# Autodesk Inventor assembly: 42146-12
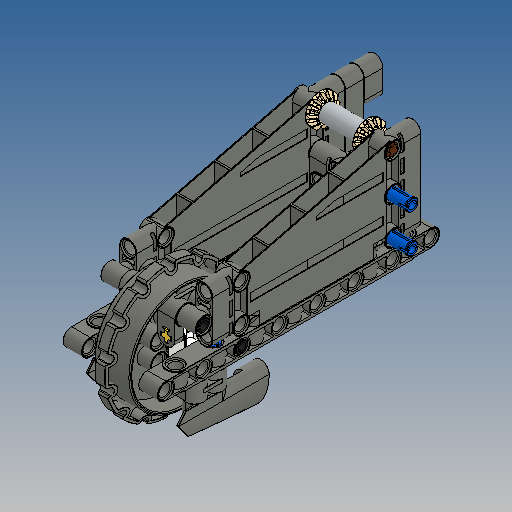
[picture p0: Inventor's stored thumbnail of the model, 512x512]
Saved by Autodesk Inventor 2025 (Build 290162010, 162A)
## iProperties
Created: 2024-11-18
Part Number: 42146-12
Material: Generisch
Document SubType Name: Assembly
Designer: hp.muther
Author: hp.muther
## Documents named in this file (20)
- D:\Inventor\Projekte\Muther\LEGO Technic\LEGO Technik - Raupenkran LR 13000 (42146)\42146-01-12.iam
- D:\Inventor\Projekte\Muther\LEGO Technic\LEGO Pieces\Paneelen\18945-DkBluishGray.ipt
- D:\Inventor\Projekte\Muther\LEGO Technic\LEGO Pieces\Pin's\2780-Black.ipt
- D:\Inventor\Projekte\Muther\LEGO Technic\LEGO Pieces\Pin's\11214-Red.ipt
- D:\Inventor\Projekte\Muther\LEGO Technic\LEGO Pieces\Pin's\6558-Blue.ipt
- D:\Inventor\Projekte\Muther\LEGO Technic\LEGO Pieces\Lochbalken\60483-DkBluishGray.ipt
- D:\Inventor\Projekte\Muther\LEGO Technic\LEGO Pieces\Lochbalken\32316-DkBluishGray.ipt
- D:\Inventor\Projekte\Muther\LEGO Technic\LEGO Pieces\Verbindungselemente\15100-DkBluishGray.ipt
- D:\Inventor\Projekte\Muther\LEGO Technic\LEGO Pieces\Achsen\4519-Yellow.ipt
- D:\Inventor\Projekte\Muther\LEGO Technic\LEGO Pieces\Verbindungselemente\41678-DkBluishGray.ipt
- D:\Inventor\Projekte\Muther\LEGO Technic\LEGO Pieces\Verbindungselemente\32184-White.ipt
- D:\Inventor\Projekte\Muther\LEGO Technic\LEGO Pieces\Achsen\24316-ReddishBrown.ipt
- D:\Inventor\Projekte\Muther\LEGO Technic\LEGO Pieces\Paneelen\11946-DkBluishGray.ipt
- D:\Inventor\Projekte\Muther\LEGO Technic\LEGO Pieces\Verbindungselemente\39793-DkBluishGray.ipt
- D:\Inventor\Projekte\Muther\LEGO Technic\LEGO Pieces\Achsen\15462-ReddishBrown.ipt
- D:\Inventor\Projekte\Muther\LEGO Technic\LEGO Pieces\Zahnrad\6589-Tan.ipt
- D:\Inventor\Projekte\Muther\LEGO Technic\LEGO Pieces\Rund\62462-LtBluishGray.ipt
- D:\Inventor\Projekte\Muther\LEGO Technic\LEGO Pieces\Lochbalken\771710-DkBluishGray.ipt
- D:\Inventor\Projekte\Muther\LEGO Technic\LEGO Pieces\Paneelen\11947-DkBluishGray.ipt
- D:\Inventor\Projekte\Muther\LEGO Technic\LEGO Pieces\Räder, Raupe\45229-DkBluishGray.ipt
## Components (48 placed, 19 different names)
1. 18945-DkBluishGray:1 — Einfügen:9, Passend:2, Einfügen:10, Einfügen:11, Einfügen:12, Einfügen:13, Winkel:1, Einfügen:29, Passend:8, Einfügen:31
2. 2780-Black:1 — Einfügen:6
3. 2780-Black:2 — Einfügen:8, Passend:2
4. 2780-Black:3 — Einfügen:11, Passend:3
5. 11214-Red:1 — Einfügen:5, Passend:1
6. 2780-Black:4 — Einfügen:12
7. 2780-Black:5 — Einfügen:14, Passend:14
8. 2780-Black:6 — Einfügen:22, Passend:7
9. 6558-Blue:1 — Einfügen:21
10. 6558-Blue:2 — Einfügen:26
11. 6558-Blue:3 — Einfügen:27
12. 6558-Blue:4 — Einfügen:28, Passend:8
13. 6558-Blue:5 — Einfügen:25, Passend:16
14. 2780-Black:7 — Einfügen:35
15. 2780-Black:8 — Einfügen:36, Passend:9
16. 2780-Black:9 — Einfügen:39, Passend:13
17. 2780-Black:10 — Einfügen:38
18. 2780-Black:11 — Einfügen:45, Passend:15
19. 6558-Blue:6 — Einfügen:44
20. 60483-DkBluishGray:1 — Einfügen:5, Einfügen:6, Einfügen:7
21. 32316-DkBluishGray:1 — Einfügen:7, Passend:1, Einfügen:8, Einfügen:9
22. 15100-DkBluishGray:1 — Einfügen:10, Einfügen:15, Winkel:1
23. 771710-DkBluishGray:1 — Einfügen:13, Passend:3, Einfügen:14, Einfügen:23
24. 2780-Black:12 — Einfügen:15
25. 4519-Yellow:1 — Einfügen:1, Passend:4, Passend:6
26. 41678-DkBluishGray:1 — Einfügen:1, Einfügen:16
27. 32184-White:1 — Einfügen:16, Passend:4, Passend:5, Einfügen:17, Einfügen:19, Passend:19
28. 4519-Yellow:2 — Passend:5
29. 41678-DkBluishGray:2 — Einfügen:17, Einfügen:18, Einfügen:23, Einfügen:24, Passend:7
30. 32184-White:2 — Einfügen:18, Passend:6, Passend:14
31. 24316-ReddishBrown:1 — Einfügen:19, Passend:17, Passend:18
32. 11946-DkBluishGray:1 — Einfügen:21, Einfügen:22, Einfügen:24
33. 39793-DkBluishGray:1 — Einfügen:25, Einfügen:26, Einfügen:27, Einfügen:28, Einfügen:29, Einfügen:47
34. 15462-ReddishBrown:1 — Einfügen:30, Einfügen:31
35. 6589-Tan:1 — Einfügen:30, Einfügen:32
36. 6589-Tan:2 — Einfügen:33
37. 62462-LtBluishGray:1 — Einfügen:32, Einfügen:33
38. 18945-DkBluishGray:2 — Einfügen:34, Winkel:2, Einfügen:35, Einfügen:36, Einfügen:37, Einfügen:47, Passend:16
39. 15100-DkBluishGray:2 — Einfügen:34, Winkel:2, Einfügen:38
40. 771710-DkBluishGray:2 — Einfügen:37, Passend:9, Einfügen:39, Einfügen:43, Pos. Zahnrad
41. 4519-Yellow:3 — Passend:10, Passend:12
42. 41678-DkBluishGray:3 — Einfügen:40
43. 4519-Yellow:4 — Passend:11
44. 41678-DkBluishGray:4 — Einfügen:41, Einfügen:42, Einfügen:43, Einfügen:46, Passend:15
45. 32184-White:4 — Einfügen:42, Passend:12, Passend:13
46. 32184-White:5 — Passend:10, Einfügen:40, Passend:11, Einfügen:41
47. 11947-DkBluishGray:1 — Einfügen:44, Einfügen:45, Einfügen:46
48. 45229-DkBluishGray:1 — Passend:17, Passend:18, Passend:19, Pos. Zahnrad
## Relationships (68: Insert 46, Mate 20, Angle 2)
- Pos. Zahnrad [Mate] (12.659 mm): 771710-DkBluishGray:2 ↔ 45229-DkBluishGray:1
- Einfügen:1 [Insert]: 4519-Yellow:1 ↔ 41678-DkBluishGray:1
- [Insert]: 4519-Yellow:2 ↔ 41678-DkBluishGray:2
- [Insert]: 4519-Yellow:3 ↔ 41678-DkBluishGray:3
- [Insert]: 4519-Yellow:4 ↔ 41678-DkBluishGray:4
- Einfügen:5 [Insert]: 11214-Red:1 ↔ 60483-DkBluishGray:1
- Einfügen:6 [Insert]: 2780-Black:1 ↔ 60483-DkBluishGray:1
- Einfügen:7 [Insert]: 60483-DkBluishGray:1 ↔ 32316-DkBluishGray:1
- Passend:1 [Mate]: 11214-Red:1 ↔ 32316-DkBluishGray:1
- Einfügen:8 [Insert]: 2780-Black:2 ↔ 32316-DkBluishGray:1
- Einfügen:9 [Insert]: 18945-DkBluishGray:1 ↔ 32316-DkBluishGray:1
- Passend:2 [Mate]: 18945-DkBluishGray:1 ↔ 2780-Black:2
- Einfügen:10 [Insert]: 18945-DkBluishGray:1 ↔ 15100-DkBluishGray:1
- Einfügen:11 [Insert]: 18945-DkBluishGray:1 ↔ 2780-Black:3
- Einfügen:12 [Insert]: 18945-DkBluishGray:1 ↔ 2780-Black:4
- Einfügen:13 [Insert]: 18945-DkBluishGray:1 ↔ 771710-DkBluishGray:1
- Passend:3 [Mate]: 2780-Black:3 ↔ 771710-DkBluishGray:1
- Einfügen:14 [Insert]: 2780-Black:5 ↔ 771710-DkBluishGray:1
- Einfügen:15 [Insert]: 15100-DkBluishGray:1 ↔ 2780-Black:12
- Einfügen:16 [Insert]: 41678-DkBluishGray:1 ↔ 32184-White:1
- Passend:4 [Mate]: 4519-Yellow:1 ↔ 32184-White:1
- Passend:5 [Mate]: 32184-White:1 ↔ 4519-Yellow:2
- Einfügen:17 [Insert]: 32184-White:1 ↔ 41678-DkBluishGray:2
- Einfügen:18 [Insert]: 41678-DkBluishGray:2 ↔ 32184-White:2
- Passend:6 [Mate]: 4519-Yellow:1 ↔ 32184-White:2
- Einfügen:19 [Insert]: 32184-White:1 ↔ 24316-ReddishBrown:1
- Winkel:1 [Angle] (0 deg): 18945-DkBluishGray:1 ↔ 15100-DkBluishGray:1
- Einfügen:21 [Insert]: 6558-Blue:1 ↔ 11946-DkBluishGray:1
- Einfügen:22 [Insert]: 2780-Black:6 ↔ 11946-DkBluishGray:1
- Einfügen:23 [Insert]: 771710-DkBluishGray:1 ↔ 41678-DkBluishGray:2
- Einfügen:24 [Insert]: 41678-DkBluishGray:2 ↔ 11946-DkBluishGray:1
- Passend:7 [Mate]: 2780-Black:6 ↔ 41678-DkBluishGray:2
- Einfügen:25 [Insert]: 6558-Blue:5 ↔ 39793-DkBluishGray:1
- Einfügen:26 [Insert]: 6558-Blue:2 ↔ 39793-DkBluishGray:1
- Einfügen:27 [Insert]: 6558-Blue:3 ↔ 39793-DkBluishGray:1
- Einfügen:28 [Insert]: 6558-Blue:4 ↔ 39793-DkBluishGray:1
- Einfügen:29 [Insert]: 18945-DkBluishGray:1 ↔ 39793-DkBluishGray:1
- Passend:8 [Mate]: 18945-DkBluishGray:1 ↔ 6558-Blue:4
- Einfügen:30 [Insert] (7.2 mm): 15462-ReddishBrown:1 ↔ 6589-Tan:1
- Einfügen:31 [Insert]: 18945-DkBluishGray:1 ↔ 15462-ReddishBrown:1
- Einfügen:32 [Insert]: 6589-Tan:1 ↔ 62462-LtBluishGray:1
- Einfügen:33 [Insert]: 6589-Tan:2 ↔ 62462-LtBluishGray:1
- Einfügen:34 [Insert]: 18945-DkBluishGray:2 ↔ 15100-DkBluishGray:2
- Winkel:2 [Angle] (0 deg): 18945-DkBluishGray:2 ↔ 15100-DkBluishGray:2
- Einfügen:35 [Insert]: 2780-Black:7 ↔ 18945-DkBluishGray:2
- Einfügen:36 [Insert]: 2780-Black:8 ↔ 18945-DkBluishGray:2
- Einfügen:37 [Insert]: 18945-DkBluishGray:2 ↔ 771710-DkBluishGray:2
- Passend:9 [Mate]: 2780-Black:8 ↔ 771710-DkBluishGray:2
- Einfügen:38 [Insert]: 2780-Black:10 ↔ 15100-DkBluishGray:2
- Einfügen:39 [Insert]: 2780-Black:9 ↔ 771710-DkBluishGray:2
- Passend:10 [Mate]: 4519-Yellow:3 ↔ 32184-White:5
- Einfügen:40 [Insert]: 41678-DkBluishGray:3 ↔ 32184-White:5
- Passend:11 [Mate]: 4519-Yellow:4 ↔ 32184-White:5
- Einfügen:41 [Insert]: 41678-DkBluishGray:4 ↔ 32184-White:5
- Einfügen:42 [Insert]: 41678-DkBluishGray:4 ↔ 32184-White:4
- Passend:12 [Mate]: 4519-Yellow:3 ↔ 32184-White:4
- Einfügen:43 [Insert]: 771710-DkBluishGray:2 ↔ 41678-DkBluishGray:4
- Passend:13 [Mate]: 2780-Black:9 ↔ 32184-White:4
- Passend:14 [Mate]: 2780-Black:5 ↔ 32184-White:2
- Einfügen:44 [Insert]: 6558-Blue:6 ↔ 11947-DkBluishGray:1
- Einfügen:45 [Insert]: 2780-Black:11 ↔ 11947-DkBluishGray:1
- Einfügen:46 [Insert]: 41678-DkBluishGray:4 ↔ 11947-DkBluishGray:1
- Passend:15 [Mate]: 2780-Black:11 ↔ 41678-DkBluishGray:4
- Einfügen:47 [Insert]: 39793-DkBluishGray:1 ↔ 18945-DkBluishGray:2
- Passend:16 [Mate]: 6558-Blue:5 ↔ 18945-DkBluishGray:2
- Passend:17 [Mate]: 24316-ReddishBrown:1 ↔ 45229-DkBluishGray:1
- Passend:18 [Mate]: 24316-ReddishBrown:1 ↔ 45229-DkBluishGray:1
- Passend:19 [Mate]: 32184-White:1 ↔ 45229-DkBluishGray:1
## Named parameters: d1_d0 = 0 mm, d2_d0 = 0 mm, d3_d1_d0 = 0 mm
